# Autodesk Inventor assembly: Assembly17
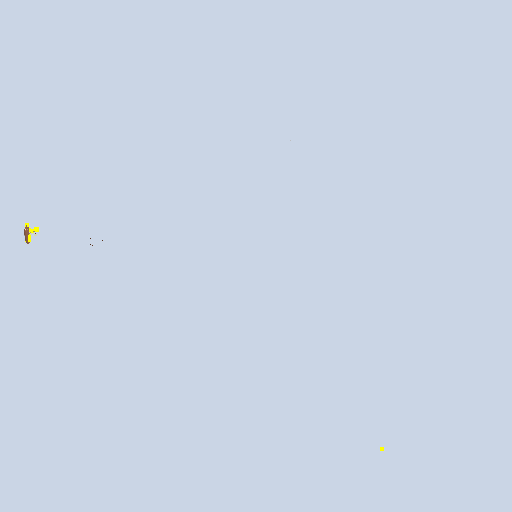
[picture p0: Inventor's stored thumbnail of the model, 512x512]
Saved by Autodesk Inventor 2024.1 (Build 281209000, 209)
## iProperties
Created: 2023-11-10
Part Number: Assembly17
Document SubType Name: Assembly
Designer: luvag
Author: luvag
## Documents named in this file (3)
- C:\Users\luvag\Desktop\Assembly17.iam
- C:\Users\luvag\Desktop\Assembly12.iam
- C:\Users\luvag\Desktop\Assembly16.iam
## Components (2 placed, 2 different names)
1. Assembly12:1 [sub-assembly]
2. Assembly16:1 [sub-assembly]
## Relationships (1: Mate 1)
- [Mate]: Assembly12:1 ↔ Assembly16:1
